# Autodesk Inventor assembly: CycloidalGear
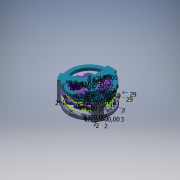
[picture p0: Inventor's stored thumbnail of the model, 180x180]
Saved by Autodesk Inventor 2018.3 (Build 223284000, 284)
## iProperties
Created: 2018-07-20
Part Number: CycloidalGear
Material: Generisch
Document SubType Name: Assembly
Designer: JochenAlt
Author: JochenAlt
## Documents named in this file (10)
- D:\Projects\FlowerPot\CAD\CycloidalGear\CycloidalGear.iam
- D:\Projects\FlowerPot\CAD\CycloidalGear\ExcentricShaft.ipt
- D:\Projects\FlowerPot\CAD\CycloidalGear\W 61700 X-2RS1.iam
- D:\Projects\FlowerPot\CAD\CycloidalGear\ShaftHolder.ipt
- D:\Projects\FlowerPot\CAD\CycloidalGear\MotorShaft.ipt
- C:\Users\JochenAlt\Documents\Inventor\Content Center Files\R2018\de-DE\DIN BEARING(1)\DIN 625 SKF - SKF 623.ipt
- D:\Projects\FlowerPot\CAD\CycloidalGear\Output.ipt
- D:\Projects\FlowerPot\CAD\CycloidalGear\Rotor.ipt
- Excenter1.ipt
- D:\Projects\FlowerPot\CAD\CycloidalGear\Rotor2.ipt
## Components (18 placed, 7 different names)
1. ExcentricShaft:3 — Passend:150, Passend:151, Passend:154, Passend:155, Passend:207, Fluchtend:6, Drehung:3
2. ExcentricShaft:6 — Passend:148, Passend:149, Passend:156, Passend:157, Passend:206, Fluchtend:5
3. ExcentricShaft:7 — Passend:146, Passend:147, Passend:152, Passend:153, Passend:208, Fluchtend:7
4. W 61700 X-2RS1:1 [sub-assembly] — Passend:179, Passend:180, Passend:217
5. W 61700 X-2RS1:2 [sub-assembly] — Passend:181, Passend:182, Fluchtend:4
6. W 61700 X-2RS1:3 [sub-assembly] — Passend:149, Passend:156
7. W 61700 X-2RS1:4 [sub-assembly] — Passend:146, Passend:152, Passend:212
8. W 61700 X-2RS1:5 [sub-assembly] — Passend:150, Passend:155, Passend:211, Fluchtend:8
9. W 61700 X-2RS1:6 [sub-assembly] — Passend:148, Passend:157, Fluchtend:4, Passend:213
10. W 61700 X-2RS1:7 [sub-assembly] — Passend:147, Passend:153, Passend:215
11. W 61700 X-2RS1:8 [sub-assembly] — Passend:151, Passend:154, Passend:214, Passend:216
12. Enclosure:1 — Passend:158, Passend:159, Passend:176, Passend:177, Passend:184, Passend:185, Passend:210
13. DIN 625 SKF SKF 623:1 — Passend:176, Passend:177, Passend:183, Passend:205, Passend:209
14. Output:1 — Drehung:2, Passend:206, Passend:207, Passend:208, Fluchtend:5, Fluchtend:6, Fluchtend:7, Passend:210
15. MotorShaft:8 — Passend:179, Passend:180, Passend:181, Passend:182, Passend:183, Drehung:2, Passend:205, Passend:209, Drehung:3
16. DIN 625 SKF SKF 623:2 — Passend:184, Passend:185
17. Excenter1:1 — Passend:211, Passend:212, Passend:213, Fluchtend:8
18. Excenter1:2 — Passend:214, Passend:215, Passend:216, Passend:217
## Relationships (43: Mate 36, Flush 5, RelateRotation 2)
- Passend:146 [Mate]: ExcentricShaft:7 ↔ W 61700 X-2RS1:4
- Passend:147 [Mate]: ExcentricShaft:7 ↔ W 61700 X-2RS1:7
- Passend:148 [Mate]: ExcentricShaft:6 ↔ W 61700 X-2RS1:6
- Passend:149 [Mate]: ExcentricShaft:6 ↔ W 61700 X-2RS1:3
- Passend:150 [Mate]: ExcentricShaft:3 ↔ W 61700 X-2RS1:5
- Passend:151 [Mate]: ExcentricShaft:3 ↔ W 61700 X-2RS1:8
- Passend:152 [Mate]: ExcentricShaft:7 ↔ W 61700 X-2RS1:4
- Passend:153 [Mate]: ExcentricShaft:7 ↔ W 61700 X-2RS1:7
- Passend:154 [Mate]: ExcentricShaft:3 ↔ W 61700 X-2RS1:8
- Passend:155 [Mate]: ExcentricShaft:3 ↔ W 61700 X-2RS1:5
- Passend:156 [Mate]: ExcentricShaft:6 ↔ W 61700 X-2RS1:3
- Passend:157 [Mate]: ExcentricShaft:6 ↔ W 61700 X-2RS1:6
- Passend:158 [Mate]: Enclosure:1
- Passend:159 [Mate]: Enclosure:1
- Passend:176 [Mate]: Enclosure:1 ↔ DIN 625 SKF SKF 623:1
- Passend:177 [Mate]: Enclosure:1 ↔ DIN 625 SKF SKF 623:1
- Passend:179 [Mate]: W 61700 X-2RS1:1 ↔ MotorShaft:8
- Passend:180 [Mate]: W 61700 X-2RS1:1 ↔ MotorShaft:8
- Passend:181 [Mate]: W 61700 X-2RS1:2 ↔ MotorShaft:8
- Passend:182 [Mate]: W 61700 X-2RS1:2 ↔ MotorShaft:8
- Passend:183 [Mate]: DIN 625 SKF SKF 623:1 ↔ MotorShaft:8
- Passend:184 [Mate]: Enclosure:1 ↔ DIN 625 SKF SKF 623:2
- Passend:185 [Mate]: Enclosure:1 ↔ DIN 625 SKF SKF 623:2
- Drehung:2 [RelateRotation] (0.0909 ul): Output:1 ↔ MotorShaft:8
- Fluchtend:4 [Flush]: W 61700 X-2RS1:2 ↔ W 61700 X-2RS1:6
- Passend:205 [Mate]: DIN 625 SKF SKF 623:1 ↔ MotorShaft:8
- Passend:206 [Mate]: ExcentricShaft:6 ↔ Output:1
- Passend:207 [Mate]: ExcentricShaft:3 ↔ Output:1
- Passend:208 [Mate]: ExcentricShaft:7 ↔ Output:1
- Fluchtend:5 [Flush]: ExcentricShaft:6 ↔ Output:1
- Passend:209 [Mate]: DIN 625 SKF SKF 623:1 ↔ MotorShaft:8
- Fluchtend:6 [Flush]: ExcentricShaft:3 ↔ Output:1
- Fluchtend:7 [Flush]: ExcentricShaft:7 ↔ Output:1
- Passend:210 [Mate]: Enclosure:1 ↔ Output:1
- Passend:211 [Mate]: W 61700 X-2RS1:5 ↔ Excenter1:1
- Passend:212 [Mate]: W 61700 X-2RS1:4 ↔ Excenter1:1
- Passend:213 [Mate]: W 61700 X-2RS1:6 ↔ Excenter1:1
- Fluchtend:8 [Flush]: W 61700 X-2RS1:5 ↔ Excenter1:1
- Passend:214 [Mate]: W 61700 X-2RS1:8 ↔ Excenter1:2
- Passend:215 [Mate]: W 61700 X-2RS1:7 ↔ Excenter1:2
- Passend:216 [Mate]: W 61700 X-2RS1:8 ↔ Excenter1:2
- Passend:217 [Mate]: W 61700 X-2RS1:1 ↔ Excenter1:2
- Drehung:3 [RelateRotation] (1 ul): ExcentricShaft:3 ↔ MotorShaft:8
